# Autodesk Inventor assembly: HbSocketU02
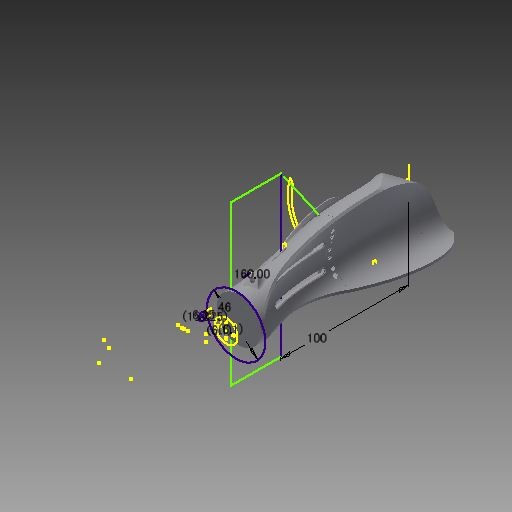
[picture p0: Inventor's stored thumbnail of the model, 512x512]
Saved by Autodesk Inventor 2018 (Build 220112000, 112)
## iProperties
Created: 2015-02-09
Part Number: HbSocketU02
Document SubType Name: Assembly
Designer: Yamaura
Author: Yamaura
## Documents named in this file (10)
- D:\cloudstrage\NextCloud\Cad_mechanical\HACKberry_sktometometo\HACKberry-hardware\3D_69%inlength\Inventor\HbSocketU02ForChild\HbSocketU02ForChild.iam
- D:\cloudstrage\NextCloud\Cad_mechanical\HACKberry_sktometometo\HACKberry-hardware\3D_69%inlength\Inventor\HbSocketU02ForChild\HbBatteryDoor03.ipt
- D:\cloudstrage\NextCloud\Cad_mechanical\HACKberry_sktometometo\HACKberry-hardware\3D_69%inlength\Inventor\HbSocketU02ForChild\HbBatteryDoorKnob03.ipt
- D:\cloudstrage\NextCloud\Cad_mechanical\HACKberry_sktometometo\HACKberry-hardware\3D_69%inlength\Inventor\HbSocketU02ForChild\HbBatteryHingeA03.ipt
- D:\cloudstrage\NextCloud\Cad_mechanical\HACKberry_sktometometo\HACKberry-hardware\3D_69%inlength\Inventor\HbSocketU02ForChild\HbBatteryHingeB03.ipt
- D:\cloudstrage\NextCloud\Cad_mechanical\HACKberry_sktometometo\HACKberry-hardware\3D_69%inlength\Inventor\HbSocketU02ForChild\HbBatteryHingeC03.ipt
- D:\cloudstrage\NextCloud\Cad_mechanical\HACKberry_sktometometo\HACKberry-hardware\3D_69%inlength\Inventor\HbSocketU02ForChild\HbBatteryDoorLever03.ipt
- D:\cloudstrage\NextCloud\Cad_mechanical\HACKberry_sktometometo\HACKberry-hardware\3D_69%inlength\Inventor\HbSocketU02ForChild\HbMainFrameA01.ipt
- D:\cloudstrage\NextCloud\Cad_mechanical\HACKberry_sktometometo\HACKberry-hardware\3D_69%inlength\Inventor\HbSocketU02ForChild\HbMainFrameB01.ipt
- D:\cloudstrage\NextCloud\Cad_mechanical\HACKberry_sktometometo\HACKberry-hardware\3D_69%inlength\Inventor\HbBatteryCase\HbBatteryCase.iam
## Components (12 placed, 9 different names)
1. HbBatteryHingeC03:1 — 挿入:6, 挿入:7
2. HbBatteryHingeB03:1 — 挿入:8, 挿入:9
3. HbBatteryHingeA03:1 — 挿入:10, 挿入:11
4. HbBatteryDoor03:1 — 挿入:6, 挿入:7, 挿入:8, 挿入:9, 挿入:10, 挿入:11, 挿入:12
5. HbMainFrameA01:1 — メイト:1, メイト:2, 挿入:4, 挿入:5
6. HbBatteryDoorKnob03:3 — メイト:1, メイト:2, 挿入:3
7. HbMainFrameB01:1 — 挿入:4, 挿入:5, 挿入:12, メイト:4
8. HbBatteryCase:1 [sub-assembly] — メイト:4
9. HbBatteryDoorKnob03:1
10. HbBatteryDoorKnob03:2
11. HbBatteryDoorLever03:1
12. HbBatteryDoorLever03:2 — 挿入:3
## Component patterns: (2 elements, first: HbBatteryDoorKnob03:1), (2 elements, first: HbBatteryDoorLever03:1)
## Relationships (13: Insert 10, Mate 3)
- メイト:1 [Mate]: HbMainFrameA01:1 ↔ HbBatteryDoorKnob03:3
- メイト:2 [Mate]: HbMainFrameA01:1 ↔ HbBatteryDoorKnob03:3
- 挿入:3 [Insert]: HbBatteryDoorKnob03:3 ↔ HbBatteryDoorLever03:2
- 挿入:4 [Insert]: HbMainFrameA01:1 ↔ HbMainFrameB01:1
- 挿入:5 [Insert]: HbMainFrameA01:1 ↔ HbMainFrameB01:1
- 挿入:6 [Insert]: HbBatteryHingeC03:1 ↔ HbBatteryDoor03:1
- 挿入:7 [Insert]: HbBatteryHingeC03:1 ↔ HbBatteryDoor03:1
- 挿入:8 [Insert]: HbBatteryHingeB03:1 ↔ HbBatteryDoor03:1
- 挿入:9 [Insert]: HbBatteryHingeB03:1 ↔ HbBatteryDoor03:1
- 挿入:10 [Insert]: HbBatteryHingeA03:1 ↔ HbBatteryDoor03:1
- 挿入:11 [Insert]: HbBatteryHingeA03:1 ↔ HbBatteryDoor03:1
- 挿入:12 [Insert]: HbBatteryDoor03:1 ↔ HbMainFrameB01:1
- メイト:4 [Mate]: HbMainFrameB01:1 ↔ HbBatteryCase:1
